# Autodesk Inventor assembly: square_alt_one
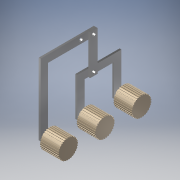
[picture p0: Inventor's stored thumbnail of the model, 180x180]
Saved by Autodesk Inventor 2018.1 (Build 221171000, 171)
## iProperties
Created: 2017-10-26
Part Number: square_alt_one
Material: 一般
Document SubType Name: Assembly
Designer: Kakeru Yamashita
Author: Kakeru Yamashita
## Documents named in this file (5)
- C:\Users\Kakeru Yamashita\Documents\Inventor\Rocker_bogie_sim\square_alt_one.iam
- C:\Users\Kakeru Yamashita\Documents\Inventor\Rocker_bogie_sim\bogie_square_alt.ipt
- C:\Users\Kakeru Yamashita\Documents\Inventor\Rocker_bogie_sim\tire.ipt
- C:\Users\Kakeru Yamashita\Documents\Inventor\Rocker_bogie_sim\rocker_bogie_plate.ipt
- C:\Users\Kakeru Yamashita\Documents\Inventor\Rocker_bogie_sim\rocker_alt.ipt
## Components (6 placed, 4 different names)
1. bogie_square_alt:1 — メイト:1, メイト:2, フラッシュ:2, メイト:6, メイト:7, フラッシュ:5, メイト:11
2. tire:1 — メイト:2, フラッシュ:1
3. tire:2 — メイト:1, フラッシュ:1, フラッシュ:2
4. tire:3 — メイト:8, フラッシュ:6
5. rocker_bogie_plate:1 — メイト:6, メイト:7, フラッシュ:5, メイト:9, メイト:10, フラッシュ:7
6. rocker_alt:1 — メイト:8, フラッシュ:6, メイト:9, メイト:10, フラッシュ:7, フラッシュ:8
## Relationships (14: Mate 8, Flush 6)
- メイト:1 [Mate]: bogie_square_alt:1 ↔ tire:2
- メイト:2 [Mate]: bogie_square_alt:1 ↔ tire:1
- フラッシュ:1 [Flush]: tire:1 ↔ tire:2
- フラッシュ:2 [Flush]: bogie_square_alt:1 ↔ tire:2
- メイト:6 [Mate]: bogie_square_alt:1 ↔ rocker_bogie_plate:1
- メイト:7 [Mate]: bogie_square_alt:1 ↔ rocker_bogie_plate:1
- フラッシュ:5 [Flush]: bogie_square_alt:1 ↔ rocker_bogie_plate:1
- メイト:8 [Mate]: tire:3 ↔ rocker_alt:1
- フラッシュ:6 [Flush]: tire:3 ↔ rocker_alt:1
- メイト:9 [Mate]: rocker_bogie_plate:1 ↔ rocker_alt:1
- メイト:10 [Mate]: rocker_bogie_plate:1 ↔ rocker_alt:1
- フラッシュ:7 [Flush]: rocker_bogie_plate:1 ↔ rocker_alt:1
- メイト:11 [Mate]: bogie_square_alt:1
- フラッシュ:8 [Flush]: rocker_alt:1
